# Autodesk Inventor assembly: XCarriageBushing
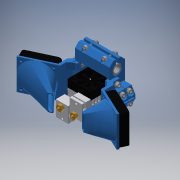
[picture p0: Inventor's stored thumbnail of the model, 180x180]
Saved by Autodesk Inventor 2016 (Build 200138000, 138)
## iProperties
Created: 2014-12-10
Part Number: XCarriageBushing
Document SubType Name: Assembly
Designer: Jack
Mass: 248.132 g
Surface Area: 960.041 cm^2
Volume: 117.803 cm^3
Density: 2.10633 g/cm^3
Author: Jack
Title: X Carriage
## Documents named in this file (15)
- C:\Users\Jack\ownCloud\Projects\CrossBot\InventorModel\XAxis\XCarriageBushing.iam
- C:\Users\Jack\ownCloud\Projects\CrossBot\InventorModel\HotEnds\E3DChimera\E3DChimera.iam
- C:\Users\Jack\ownCloud\Projects\CrossBot\InventorModel\Electronics\EndStops\EndStopOptical.ipt
- C:\Users\Jack\ownCloud\Projects\CrossBot\InventorModel\XAxis\XCarriageBeltClipRound.ipt
- C:\Users\Jack\ownCloud\Projects\CrossBot\InventorModel\Hardware\Nuts\Nut3.ipt
- C:\Users\Jack\ownCloud\Projects\CrossBot\InventorModel\Hardware\BoltWashers\BoltWasher3\BoltWasher3x16.iam
- C:\Users\Jack\ownCloud\Projects\CrossBot\InventorModel\Hardware\Bolts\SHCS\SHCS3\SHCS3x10.ipt
- C:\Users\Jack\ownCloud\Projects\CrossBot\InventorModel\Electronics\Fans\Fan40mm.ipt
- C:\Users\Jack\ownCloud\Projects\CrossBot\InventorModel\Hardware\BoltWashers\BoltWasher3\BoltWasher3x10.iam
- C:\Users\Jack\ownCloud\Projects\CrossBot\InventorModel\XAxis\ChimeraXCarriage5FanDuct2.ipt
- C:\Users\Jack\ownCloud\Projects\CrossBot\InventorModel\XAxis\ChimeraXCarriage5FanDuct2Mirrored.ipt
- C:\Users\Jack\ownCloud\Projects\CrossBot\InventorModel\Hardware\BoltWashers\BoltWasher3\BoltWasher3x8.iam
- C:\Users\Jack\ownCloud\Projects\CrossBot\InventorModel\XAxis\ChimeraXCarriageBushings.ipt
- C:\Users\Jack\ownCloud\Projects\CrossBot\InventorModel\Hardware\BoltWashers\BoltWasher3\BoltWasher3x14.iam
- C:\Users\Jack\ownCloud\Projects\CrossBot\InventorModel\Hardware\Bearing\BearingLinear\BearingLinearPlastic\BearingPlastic8x12x12.ipt
## Components (54 placed, 14 different names)
1. E3DChimera:1 [sub-assembly] — Mate:257, Mate:258, Mate:259, Mate:260
2. EndStopOptical:1 — Mate:195, Mate:196, Mate:197, Mate:198, Mate:295
3. XCarriageBeltClipRound:1 — Mate:41, Mate:43, Mate:53, Mate:56, Mate:324
4. XCarriageBeltClipRound:2 — Mate:42, Mate:44, Mate:54, Mate:55, Mate:325
5. XCarriageBeltClipRound:3 — Mate:45, Mate:47, Mate:49, Mate:51, Mate:322
6. XCarriageBeltClipRound:4 — Mate:46, Mate:48, Mate:50, Mate:52, Mate:323
7. ChimeraXCarriage5FanDuct2:1 — Mate:225, Mate:228, Mate:229, Mate:231, Mate:232, Mate:233, Mate:250, Mate:316
8. ChimeraXCarriage5FanDuct2Mirrored:1 — Mate:234, Mate:235, Mate:236, Mate:237, Mate:241, Mate:242, Mate:243, Mate:317
9. BoltWasher3x8:1 [sub-assembly] — Mate:286, Mate:289
10. BoltWasher3x8:2 [sub-assembly] — Mate:285, Mate:290
11. BoltWasher3x8:3 [sub-assembly] — Mate:287, Mate:288
12. ChimeraXCarriageBushings:1 — Mate:257, Mate:258, Mate:259, Mate:260, Angle:1, Angle:2, Angle:3, Angle:4, Mate:269, Mate:270, Mate:271, Mate:272, Mate:273, Mate:274, Mate:275, Mate:276, Mate:277, Mate:278, Mate:279, Mate:280, Mate:285, Mate:286, Mate:287, Mate:288, Mate:289, Mate:290, Mate:291, Mate:292, Mate:293, Mate:294, Angle:5, Angle:6, Mate:295, Mate:296, Mate:297, Mate:298, Mate:299, Mate:300, Mate:301, Mate:302, Mate:303, Angle:7, Angle:8, Mate:304, Mate:305, Angle:9, Angle:10, Mate:306, Mate:307, Angle:11, Angle:12, Mate:308, Mate:309, Angle:13, Angle:14, Mate:310, Mate:311, Mate:312, Mate:313, Mate:314, Mate:315, Mate:316, Mate:317, Angle:15, Angle:16, Angle:17, Mate:318, Mate:319, Mate:320, Angle:18, Mate:321, Mate:322, Mate:323, Mate:324, Mate:325, Mate:326, Mate:327, Mate:328, Mate:329, Flush:1, Flush:2, Flush:3, Flush:4
13. BoltWasher3x14:1 [sub-assembly] — Mate:274, Mate:279, Mate:282
14. BoltWasher3x14:2 [sub-assembly] — Mate:275, Mate:278, Mate:284
15. BoltWasher3x14:3 [sub-assembly] — Mate:276, Mate:277, Mate:283
16. BoltWasher3x14:4 [sub-assembly] — Mate:273, Mate:280, Mate:281
17. BearingPlastic8x12x12:1 — Mate:329, Flush:1
18. BearingPlastic8x12x12:2 — Mate:326, Flush:3
19. BearingPlastic8x12x12:3 — Mate:328, Flush:2
20. BearingPlastic8x12x12:4 — Mate:327, Flush:4
21. Fan40mm:3 — Mate:231, Mate:232, Mate:233
22. Fan40mm:2 — Mate:241, Mate:242, Mate:243
23. Nut3:12 — Angle:1, Mate:271, Mate:283
24. Nut3:13 — Angle:2, Mate:272, Mate:284
25. Nut3:9 — Angle:3, Mate:270, Mate:281
26. Nut3:10 — Angle:4, Mate:269, Mate:282
27. BoltWasher3x16:1 [sub-assembly] — Mate:42, Mate:55, Mate:130, Mate:299
28. BoltWasher3x16:2 [sub-assembly] — Mate:41, Mate:56, Mate:128, Mate:297
29. BoltWasher3x16:3 [sub-assembly] — Mate:43, Mate:53, Mate:127, Mate:296
30. BoltWasher3x16:4 [sub-assembly] — Mate:44, Mate:54, Mate:129, Mate:298
31. BoltWasher3x16:5 [sub-assembly] — Mate:45, Mate:49, Mate:142, Mate:302
32. BoltWasher3x16:6 [sub-assembly] — Mate:46, Mate:50, Mate:144, Mate:300
33. BoltWasher3x16:7 [sub-assembly] — Mate:47, Mate:51, Mate:141, Mate:303
34. BoltWasher3x16:8 [sub-assembly] — Mate:48, Mate:52, Mate:143, Mate:301
35. Nut3:1 — Mate:141, Angle:8, Mate:304
36. Nut3:2 — Mate:143, Angle:14, Mate:310
37. Nut3:3 — Mate:127, Angle:10, Mate:306
38. Nut3:4 — Mate:129, Angle:11, Mate:309
39. Nut3:5 — Mate:142, Angle:7, Mate:305
40. Nut3:6 — Mate:144, Angle:13, Mate:311
41. Nut3:7 — Mate:128, Angle:9, Mate:307
42. Nut3:8 — Mate:130, Angle:12, Mate:308
43. Nut3:17 — Mate:218, Angle:17, Mate:318
44. BoltWasher3x10:3 [sub-assembly] — Mate:218, Mate:225, Mate:228, Mate:315
45. BoltWasher3x10:4 [sub-assembly] — Mate:217, Mate:229, Mate:250, Mate:314
46. Nut3:19 — Mate:217, Angle:16, Mate:319
47. Nut3:18 — Mate:219, Angle:18, Mate:321
48. BoltWasher3x10:2 [sub-assembly] — Mate:219, Mate:234, Mate:237, Mate:312
49. BoltWasher3x10:1 [sub-assembly] — Mate:220, Mate:235, Mate:236, Mate:313
50. Nut3:20 — Mate:220, Angle:15, Mate:320
51. SHCS3x10:2 — Mate:196, Mate:197, Mate:256, Mate:292
52. SHCS3x10:1 — Mate:195, Mate:198, Mate:252, Mate:291
53. Nut3:15 — Mate:256, Mate:293, Angle:6
54. Nut3:16 — Mate:252, Mate:294, Angle:5
## Relationships (135: Mate 113, Angle 18, Flush 4)
- Mate:41: XCarriageBeltClipRound:1 ↔ BoltWasher3x16:2
- Mate:42: XCarriageBeltClipRound:2 ↔ BoltWasher3x16:1
- Mate:43: XCarriageBeltClipRound:1 ↔ BoltWasher3x16:3
- Mate:44: XCarriageBeltClipRound:2 ↔ BoltWasher3x16:4
- Mate:45: XCarriageBeltClipRound:3 ↔ BoltWasher3x16:5
- Mate:46: XCarriageBeltClipRound:4 ↔ BoltWasher3x16:6
- Mate:47: XCarriageBeltClipRound:3 ↔ BoltWasher3x16:7
- Mate:48: XCarriageBeltClipRound:4 ↔ BoltWasher3x16:8
- Mate:49: XCarriageBeltClipRound:3 ↔ BoltWasher3x16:5
- Mate:50: XCarriageBeltClipRound:4 ↔ BoltWasher3x16:6
- Mate:51: XCarriageBeltClipRound:3 ↔ BoltWasher3x16:7
- Mate:52: XCarriageBeltClipRound:4 ↔ BoltWasher3x16:8
- Mate:53: XCarriageBeltClipRound:1 ↔ BoltWasher3x16:3
- Mate:54: XCarriageBeltClipRound:2 ↔ BoltWasher3x16:4
- Mate:55: XCarriageBeltClipRound:2 ↔ BoltWasher3x16:1
- Mate:56: XCarriageBeltClipRound:1 ↔ BoltWasher3x16:2
- Mate:127: BoltWasher3x16:3 ↔ Nut3:3
- Mate:128: BoltWasher3x16:2 ↔ Nut3:7
- Mate:129: BoltWasher3x16:4 ↔ Nut3:4
- Mate:130: BoltWasher3x16:1 ↔ Nut3:8
- Mate:141: BoltWasher3x16:7 ↔ Nut3:1
- Mate:142: BoltWasher3x16:5 ↔ Nut3:5
- Mate:143: BoltWasher3x16:8 ↔ Nut3:2
- Mate:144: BoltWasher3x16:6 ↔ Nut3:6
- Mate:195: EndStopOptical:1 ↔ SHCS3x10:1
- Mate:196: EndStopOptical:1 ↔ SHCS3x10:2
- Mate:197: EndStopOptical:1 ↔ SHCS3x10:2
- Mate:198: EndStopOptical:1 ↔ SHCS3x10:1
- Mate:217: BoltWasher3x10:4 ↔ Nut3:19
- Mate:218: Nut3:17 ↔ BoltWasher3x10:3
- Mate:219: Nut3:18 ↔ BoltWasher3x10:2
- Mate:220: BoltWasher3x10:1 ↔ Nut3:20
- Mate:225: ChimeraXCarriage5FanDuct2:1 ↔ BoltWasher3x10:3
- Mate:228: ChimeraXCarriage5FanDuct2:1 ↔ BoltWasher3x10:3
- Mate:229: ChimeraXCarriage5FanDuct2:1 ↔ BoltWasher3x10:4
- Mate:231: ChimeraXCarriage5FanDuct2:1 ↔ Fan40mm:3
- Mate:232: ChimeraXCarriage5FanDuct2:1 ↔ Fan40mm:3
- Mate:233: ChimeraXCarriage5FanDuct2:1 ↔ Fan40mm:3
- Mate:234: ChimeraXCarriage5FanDuct2Mirrored:1 ↔ BoltWasher3x10:2
- Mate:235: ChimeraXCarriage5FanDuct2Mirrored:1 ↔ BoltWasher3x10:1
- Mate:236: ChimeraXCarriage5FanDuct2Mirrored:1 ↔ BoltWasher3x10:1
- Mate:237: ChimeraXCarriage5FanDuct2Mirrored:1 ↔ BoltWasher3x10:2
- Mate:241: ChimeraXCarriage5FanDuct2Mirrored:1 ↔ Fan40mm:2
- Mate:242: ChimeraXCarriage5FanDuct2Mirrored:1 ↔ Fan40mm:2
- Mate:243: ChimeraXCarriage5FanDuct2Mirrored:1 ↔ Fan40mm:2
- Mate:250: ChimeraXCarriage5FanDuct2:1 ↔ BoltWasher3x10:4
- Mate:252: SHCS3x10:1 ↔ Nut3:16
- Mate:256: SHCS3x10:2 ↔ Nut3:15
- Mate:257: E3DChimera:1 ↔ ChimeraXCarriageBushings:1
- Mate:258: E3DChimera:1 ↔ ChimeraXCarriageBushings:1
- Mate:259: E3DChimera:1 ↔ ChimeraXCarriageBushings:1
- Mate:260: E3DChimera:1 ↔ ChimeraXCarriageBushings:1
- Angle:1 (0 deg): ChimeraXCarriageBushings:1 ↔ Nut3:12
- Angle:2 (0 deg): ChimeraXCarriageBushings:1 ↔ Nut3:13
- Angle:3 (0 deg): ChimeraXCarriageBushings:1 ↔ Nut3:9
- Angle:4 (0 deg): ChimeraXCarriageBushings:1 ↔ Nut3:10
- Mate:269: ChimeraXCarriageBushings:1 ↔ Nut3:10
- Mate:270: ChimeraXCarriageBushings:1 ↔ Nut3:9
- Mate:271: ChimeraXCarriageBushings:1 ↔ Nut3:12
- Mate:272: ChimeraXCarriageBushings:1 ↔ Nut3:13
- Mate:273: ChimeraXCarriageBushings:1 ↔ BoltWasher3x14:4
- Mate:274: ChimeraXCarriageBushings:1 ↔ BoltWasher3x14:1
- Mate:275: ChimeraXCarriageBushings:1 ↔ BoltWasher3x14:2
- Mate:276: ChimeraXCarriageBushings:1 ↔ BoltWasher3x14:3
- Mate:277: ChimeraXCarriageBushings:1 ↔ BoltWasher3x14:3
- Mate:278: ChimeraXCarriageBushings:1 ↔ BoltWasher3x14:2
- Mate:279: ChimeraXCarriageBushings:1 ↔ BoltWasher3x14:1
- Mate:280: ChimeraXCarriageBushings:1 ↔ BoltWasher3x14:4
- Mate:281: BoltWasher3x14:4 ↔ Nut3:9
- Mate:282: BoltWasher3x14:1 ↔ Nut3:10
- Mate:283: BoltWasher3x14:3 ↔ Nut3:12
- Mate:284: BoltWasher3x14:2 ↔ Nut3:13
- Mate:285: BoltWasher3x8:2 ↔ ChimeraXCarriageBushings:1
- Mate:286: BoltWasher3x8:1 ↔ ChimeraXCarriageBushings:1
- Mate:287: BoltWasher3x8:3 ↔ ChimeraXCarriageBushings:1
- Mate:288: BoltWasher3x8:3 ↔ ChimeraXCarriageBushings:1
- Mate:289: BoltWasher3x8:1 ↔ ChimeraXCarriageBushings:1
- Mate:290: BoltWasher3x8:2 ↔ ChimeraXCarriageBushings:1
- Mate:291: ChimeraXCarriageBushings:1 ↔ SHCS3x10:1
- Mate:292: ChimeraXCarriageBushings:1 ↔ SHCS3x10:2
- Mate:293: ChimeraXCarriageBushings:1 ↔ Nut3:15
- Mate:294: ChimeraXCarriageBushings:1 ↔ Nut3:16
- Angle:5 (0 deg): ChimeraXCarriageBushings:1 ↔ Nut3:16
- Angle:6 (0 deg): ChimeraXCarriageBushings:1 ↔ Nut3:15
- Mate:295 (0.5 mm): EndStopOptical:1 ↔ ChimeraXCarriageBushings:1
- Mate:296: ChimeraXCarriageBushings:1 ↔ BoltWasher3x16:3
- Mate:297: ChimeraXCarriageBushings:1 ↔ BoltWasher3x16:2
- Mate:298: ChimeraXCarriageBushings:1 ↔ BoltWasher3x16:4
- Mate:299: ChimeraXCarriageBushings:1 ↔ BoltWasher3x16:1
- Mate:300: ChimeraXCarriageBushings:1 ↔ BoltWasher3x16:6
- Mate:301: ChimeraXCarriageBushings:1 ↔ BoltWasher3x16:8
- Mate:302: ChimeraXCarriageBushings:1 ↔ BoltWasher3x16:5
- Mate:303: ChimeraXCarriageBushings:1 ↔ BoltWasher3x16:7
- Angle:7 (0 deg): ChimeraXCarriageBushings:1 ↔ Nut3:5
- Angle:8 (0 deg): ChimeraXCarriageBushings:1 ↔ Nut3:1
- Mate:304: ChimeraXCarriageBushings:1 ↔ Nut3:1
- Mate:305: ChimeraXCarriageBushings:1 ↔ Nut3:5
- Angle:9 (0 deg): ChimeraXCarriageBushings:1 ↔ Nut3:7
- Angle:10 (0 deg): ChimeraXCarriageBushings:1 ↔ Nut3:3
- Mate:306: ChimeraXCarriageBushings:1 ↔ Nut3:3
- Mate:307: ChimeraXCarriageBushings:1 ↔ Nut3:7
- Angle:11 (0 deg): ChimeraXCarriageBushings:1 ↔ Nut3:4
- Angle:12 (0 deg): ChimeraXCarriageBushings:1 ↔ Nut3:8
- Mate:308: ChimeraXCarriageBushings:1 ↔ Nut3:8
- Mate:309: ChimeraXCarriageBushings:1 ↔ Nut3:4
- Angle:13 (0 deg): ChimeraXCarriageBushings:1 ↔ Nut3:6
- Angle:14 (0 deg): ChimeraXCarriageBushings:1 ↔ Nut3:2
- Mate:310: ChimeraXCarriageBushings:1 ↔ Nut3:2
- Mate:311: ChimeraXCarriageBushings:1 ↔ Nut3:6
- Mate:312: ChimeraXCarriageBushings:1 ↔ BoltWasher3x10:2
- Mate:313: ChimeraXCarriageBushings:1 ↔ BoltWasher3x10:1
- Mate:314: ChimeraXCarriageBushings:1 ↔ BoltWasher3x10:4
- Mate:315: ChimeraXCarriageBushings:1 ↔ BoltWasher3x10:3
- Mate:316: ChimeraXCarriage5FanDuct2:1 ↔ ChimeraXCarriageBushings:1
- Mate:317: ChimeraXCarriage5FanDuct2Mirrored:1 ↔ ChimeraXCarriageBushings:1
- Angle:15 (0 deg): ChimeraXCarriageBushings:1 ↔ Nut3:20
- Angle:16 (0 deg): ChimeraXCarriageBushings:1 ↔ Nut3:19
- Angle:17 (0 deg): ChimeraXCarriageBushings:1 ↔ Nut3:17
- Mate:318: ChimeraXCarriageBushings:1 ↔ Nut3:17
- Mate:319: ChimeraXCarriageBushings:1 ↔ Nut3:19
- Mate:320: ChimeraXCarriageBushings:1 ↔ Nut3:20
- Angle:18 (0 deg): ChimeraXCarriageBushings:1 ↔ Nut3:18
- Mate:321: ChimeraXCarriageBushings:1 ↔ Nut3:18
- Mate:322: XCarriageBeltClipRound:3 ↔ ChimeraXCarriageBushings:1
- Mate:323: XCarriageBeltClipRound:4 ↔ ChimeraXCarriageBushings:1
- Mate:324: XCarriageBeltClipRound:1 ↔ ChimeraXCarriageBushings:1
- Mate:325: XCarriageBeltClipRound:2 ↔ ChimeraXCarriageBushings:1
- Mate:326: ChimeraXCarriageBushings:1 ↔ BearingPlastic8x12x12:2
- Mate:327: ChimeraXCarriageBushings:1 ↔ BearingPlastic8x12x12:4
- Mate:328: ChimeraXCarriageBushings:1 ↔ BearingPlastic8x12x12:3
- Mate:329: ChimeraXCarriageBushings:1 ↔ BearingPlastic8x12x12:1
- Flush:1: ChimeraXCarriageBushings:1 ↔ BearingPlastic8x12x12:1
- Flush:2: ChimeraXCarriageBushings:1 ↔ BearingPlastic8x12x12:3
- Flush:3: ChimeraXCarriageBushings:1 ↔ BearingPlastic8x12x12:2
- Flush:4: ChimeraXCarriageBushings:1 ↔ BearingPlastic8x12x12:4
